# Autodesk Inventor assembly: X_CarriageR_V2_1
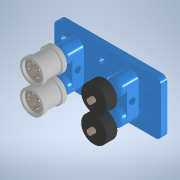
[picture p0: Inventor's stored thumbnail of the model, 180x180]
Saved by Autodesk Inventor 2022 (Build 260153000, 153)
## iProperties
Created: 2021-06-13
Part Number: X_CarriageR_V2_1
Document SubType Name: Assembly
Designer: Jorian Brusind
Author: Jorian Brusind
## Documents named in this file (10)
- C:\Users\Jorian Brusind\Documents\GitHub\HyperRail\Inventor Files\X_CarriageR_V2_1.iam
- C:\Users\Jorian Brusind\Documents\GitHub\HyperRail\Inventor Files\X_Carriage_Plate.ipt
- C:\Users\Jorian Brusind\Documents\GitHub\HyperRail\Inventor Files\4mm_Roller_Spacer_extended.ipt
- C:\Users\Jorian Brusind\Documents\GitHub\HyperRail\Inventor Files\11mm_BearingWheel.ipt
- C:\Users\Jorian Brusind\Documents\GitHub\HyperRail\Inventor Files\Bearing_Spacer.ipt
- C:\Users\Jorian Brusind\Documents\GitHub\HyperRail\Inventor Files\miniature-ball-bearings-metric-series-flanged-1.snapshot.1\F606ZZFlanged\F608 - 8 x 22 x 7.ipt
- C:\Users\Jorian Brusind\Documents\GitHub\PersonalProjects\HyperRail\Inventor Files\miniature-ball-bearings-metric-series-flanged-1.snapshot.1\F606ZZFlanged.ipt
- C:\Users\Jorian Brusind\Documents\GitHub\HyperRail\Inventor Files\685ZZFlanged_Adapter.ipt
- C:\Users\Jorian Brusind\Documents\GitHub\HyperRail\Inventor Files\Metric bolt\Bolt M5 45mm.ipt
- C:\Users\Jorian Brusind\Documents\GitHub\HyperRail\Inventor Files\Metric bolt\Bolt M5 50mm.ipt
## Components (19 placed, 8 different names)
1. X_Carriage_Plate:1 — Mate:69, Mate:72, Mate:84, Mate:85, Angle:1, Angle:2, Mate:110
2. 4mm_Roller_Spacer_extended:1 — Mate:72, Mate:74, Mate:75, Mate:76, Mate:85, Angle:1, Mate:108, Mate:109
3. 4mm_Roller_Spacer_extended:3 — Mate:69, Mate:84, Angle:2, Mate:95, Mate:96, Mate:97, Mate:111, Mate:112
4. 11mm_BearingWheel:1 — Mate:75, Flush:1, Mate:76
5. 11mm_BearingWheel:2 — Mate:74, Flush:1
6. Bearing_Spacer:1 — Flush:3, Mate:92, Mate:93, Mate:94
7. Bearing_Spacer:2 — Flush:3, Mate:89, Mate:90, Mate:91
8. F608 - 8 x 22 x 7:1 — Mate:92, Mate:94, Mate:96, Mate:99, Mate:101
9. F608 - 8 x 22 x 7:2 — Mate:93, Mate:100
10. F608 - 8 x 22 x 7:3 — Mate:90, Mate:103, Mate:105
11. F608 - 8 x 22 x 7:4 — Mate:89, Mate:91, Mate:95, Mate:97, Mate:104
12. 685ZZFlanged_Adapter:1 — Mate:99, Mate:101
13. 685ZZFlanged_Adapter:2 — Mate:100
14. 685ZZFlanged_Adapter:3 — Mate:103, Mate:105
15. 685ZZFlanged_Adapter:4 — Mate:104
16. Bolt M5 45mm:3 — Mate:109
17. Bolt M5 45mm:4 — Mate:108, Mate:110, Flush:6
18. Bolt M5 50mm:1 — Mate:111, Flush:6, Flush:7
19. Bolt M5 50mm:2 — Mate:112, Flush:7
## Relationships (38: Mate 31, Flush 5, Angle 2)
- Mate:69: X_Carriage_Plate:1 ↔ 4mm_Roller_Spacer_extended:3
- Mate:72: X_Carriage_Plate:1 ↔ 4mm_Roller_Spacer_extended:1
- Mate:74: 4mm_Roller_Spacer_extended:1 ↔ 11mm_BearingWheel:2
- Mate:75: 4mm_Roller_Spacer_extended:1 ↔ 11mm_BearingWheel:1
- Flush:1: 11mm_BearingWheel:1 ↔ 11mm_BearingWheel:2
- Mate:76: 4mm_Roller_Spacer_extended:1 ↔ 11mm_BearingWheel:1
- Mate:84 (-12.5 mm): X_Carriage_Plate:1 ↔ 4mm_Roller_Spacer_extended:3
- Mate:85 (-12.5 mm): X_Carriage_Plate:1 ↔ 4mm_Roller_Spacer_extended:1
- Angle:1 (0 deg): X_Carriage_Plate:1 ↔ 4mm_Roller_Spacer_extended:1
- Angle:2 (0 deg): X_Carriage_Plate:1 ↔ 4mm_Roller_Spacer_extended:3
- Flush:3: Bearing_Spacer:1 ↔ Bearing_Spacer:2
- [Mate]: F608 - 8 x 22 x 7:1 ↔ F608 - 8 x 22 x 7:2
- [Mate]: F608 - 8 x 22 x 7:3 ↔ F608 - 8 x 22 x 7:4
- Mate:89: Bearing_Spacer:2 ↔ F608 - 8 x 22 x 7:4
- Mate:90: Bearing_Spacer:2 ↔ F608 - 8 x 22 x 7:3
- Mate:91: Bearing_Spacer:2 ↔ F608 - 8 x 22 x 7:4
- Mate:92: Bearing_Spacer:1 ↔ F608 - 8 x 22 x 7:1
- Mate:93: Bearing_Spacer:1 ↔ F608 - 8 x 22 x 7:2
- Mate:94: Bearing_Spacer:1 ↔ F608 - 8 x 22 x 7:1
- Mate:95: 4mm_Roller_Spacer_extended:3 ↔ F608 - 8 x 22 x 7:4
- Mate:96: 4mm_Roller_Spacer_extended:3 ↔ F608 - 8 x 22 x 7:1
- Mate:97: 4mm_Roller_Spacer_extended:3 ↔ F608 - 8 x 22 x 7:4
- [Mate]: 685ZZFlanged_Adapter:1 ↔ 685ZZFlanged_Adapter:2
- Mate:99: F608 - 8 x 22 x 7:1 ↔ 685ZZFlanged_Adapter:1
- Mate:100: F608 - 8 x 22 x 7:2 ↔ 685ZZFlanged_Adapter:2
- Mate:101: F608 - 8 x 22 x 7:1 ↔ 685ZZFlanged_Adapter:1
- [Mate]: 685ZZFlanged_Adapter:3 ↔ 685ZZFlanged_Adapter:4
- Mate:103: F608 - 8 x 22 x 7:3 ↔ 685ZZFlanged_Adapter:3
- Mate:104: F608 - 8 x 22 x 7:4 ↔ 685ZZFlanged_Adapter:4
- Mate:105: F608 - 8 x 22 x 7:3 ↔ 685ZZFlanged_Adapter:3
- [Flush]: Bolt M5 45mm:3 ↔ Bolt M5 45mm:4
- Mate:108: 4mm_Roller_Spacer_extended:1 ↔ Bolt M5 45mm:4
- Mate:109: 4mm_Roller_Spacer_extended:1 ↔ Bolt M5 45mm:3
- Mate:110: X_Carriage_Plate:1 ↔ Bolt M5 45mm:4
- Mate:111: 4mm_Roller_Spacer_extended:3 ↔ Bolt M5 50mm:1
- Mate:112: 4mm_Roller_Spacer_extended:3 ↔ Bolt M5 50mm:2
- Flush:6: Bolt M5 45mm:4 ↔ Bolt M5 50mm:1
- Flush:7: Bolt M5 50mm:1 ↔ Bolt M5 50mm:2
## Named parameters: d136_d94 = 0 mm, d151_d153 = 0 mm, d157_d131 = 0 mm
